# Autodesk Inventor assembly: Assembly1
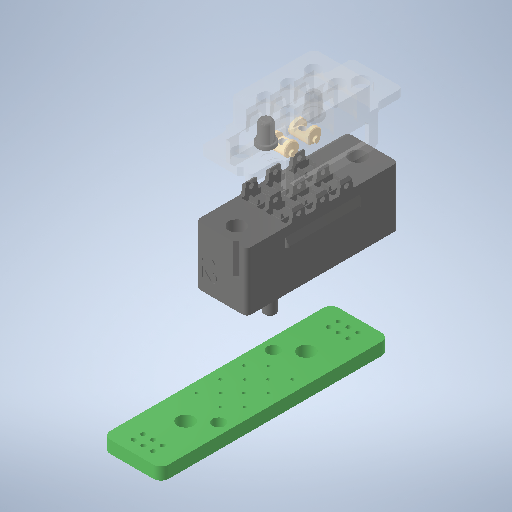
[picture p0: Inventor's stored thumbnail of the model, 512x512]
Saved by Autodesk Inventor 2025.1 (Build 291241000, 241)
## iProperties
Created: 2025-02-18
Part Number: Assembly1
Document SubType Name: Assembly
Designer: santiago
Author: santiago
## Documents named in this file (6)
- C:\Users\santiago\Documents\Tesis\3d models\scaled\Braille_assembly.iam
- C:\Users\santiago\Documents\Tesis\3d models\scaled\cam.ipt
- C:\Users\santiago\Documents\Tesis\3d models\scaled\dot.ipt
- C:\Users\santiago\Documents\Tesis\3d models\scaled\pcb.ipt
- C:\Users\santiago\Documents\Tesis\3d models\scaled\upper.ipt
- C:\Users\santiago\Documents\Tesis\3d models\scaled\lower.ipt
## Components (7 placed, 5 different names)
1. cam:1
2. dot:1 — Mate:9
3. pcb:1
4. upper:1 — Mate:9, Mate:10
5. cam:2
6. dot:2 — Mate:10
7. lower:1
## Relationships (2: Mate 2)
- Mate:9: dot:1 ↔ upper:1
- Mate:10: upper:1 ↔ dot:2
